# Autodesk Inventor assembly: Estructura_bk03
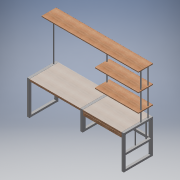
[picture p0: Inventor's stored thumbnail of the model, 180x180]
Saved by Autodesk Inventor 2016 (Build 200138000, 138)
## iProperties
Created: 2018-06-24
Part Number: Estructura_bk03
Document SubType Name: Weldment
Designer: damia
Weld Material: Iron, Cast
Mass: 65449.7 g
Surface Area: 113018 cm^2
Volume: 51991 cm^3
Density: 1.25887 g/cm^3
_SolveAssemblyDoc: Frame Generator Solve Assembly
_Version: 15.0.0
Author: damia
## Documents named in this file (12)
- C:\Users\damia\Documents\Inventor\escritorio_Damian\Estructura_bk03.iam
- C:\Users\damia\Documents\Inventor\Escritorio_Damian\Esqueleto.ipt
- C:\Users\damia\Documents\Inventor\Escritorio_Damian\Estructura\Frame\Frame0002.iam
- C:\Users\damia\Documents\Inventor\Escritorio_Damian\Part42.ipt
- C:\Users\damia\Documents\Inventor\Escritorio_Damian\VidrioChico.ipt
- C:\Users\damia\Documents\Inventor\Escritorio_Damian\tablero_chico.ipt
- C:\Users\damia\Documents\Inventor\Escritorio_Damian\tablero_granded.ipt
- C:\Users\damia\Documents\Inventor\Escritorio_Damian\Esqueleto_Estantes.ipt
- C:\Users\damia\Documents\Inventor\Escritorio_Damian\Estante01.ipt
- C:\Users\damia\Documents\Inventor\Escritorio_Damian\estante02.ipt
- C:\Users\damia\Documents\Inventor\Escritorio_Damian\FrenteChico.ipt
- C:\Users\damia\Documents\Inventor\Escritorio_Damian\FrenteGrande.ipt
## Components (13 placed, 11 different names)
1. Esqueleto:1 — Mate:1, Mate:2
2. Frame0002:1 [sub-assembly] — Flush:7, Flush:8, Flush:9, Mate:7, Flush:12, Mate:9
3. tablero_granded:1
4. tablero_chico:1
5. VidrioGrande:1
6. VidrioChico:1
7. Esqueleto_Estantes:1 — Flush:7, Flush:8
8. Estante01:1 — Flush:9, Flush:10, Flush:11
9. Estante01:2 — Flush:10, Flush:11, Mate:7
10. estante02:1 — Flush:12
11. FrenteChico:1 — Mate:10
12. FrenteGrande:1 — Flush:13, Mate:8, Mate:9, Mate:10
13. FrenteGrande:2 — Flush:13, Mate:8
## Relationships (23: Flush 13, Mate 10)
- Mate:1: Esqueleto:1
- Mate:2: Esqueleto:1
- [Flush]: tablero_granded:1 ↔ VidrioGrande:1
- [Flush]: tablero_granded:1 ↔ VidrioGrande:1
- [Flush]: tablero_chico:1 ↔ VidrioChico:1
- [Flush]: tablero_chico:1 ↔ VidrioChico:1
- [Flush]: Frame0002:1 ↔ tablero_chico:1
- [Mate]: Frame0002:1 ↔ tablero_chico:1
- [Mate]: Frame0002:1 ↔ tablero_chico:1
- [Mate]: Frame0002:1 ↔ tablero_granded:1
- [Flush]: Frame0002:1 ↔ tablero_granded:1
- [Mate]: Frame0002:1 ↔ tablero_granded:1
- Flush:7: Frame0002:1 ↔ Esqueleto_Estantes:1
- Flush:8: Frame0002:1 ↔ Esqueleto_Estantes:1
- Flush:9: Frame0002:1 ↔ Estante01:1
- Flush:10: Estante01:1 ↔ Estante01:2
- Flush:11: Estante01:1 ↔ Estante01:2
- Mate:7: Frame0002:1 ↔ Estante01:2
- Flush:12: Frame0002:1 ↔ estante02:1
- Flush:13: FrenteGrande:1 ↔ FrenteGrande:2
- Mate:8 (5 mm): FrenteGrande:1 ↔ FrenteGrande:2
- Mate:9 (5 mm): Frame0002:1 ↔ FrenteGrande:1
- Mate:10 (5 mm): FrenteChico:1 ↔ FrenteGrande:1
## Named parameters: d14_d8 = 0 mm, d16_d6 = 0 mm, d17_d7 = 0 mm, Altura = 700 mm, Profundidad = 600 mm, TablaAltura = 40 mm, CajonAltura = 370 mm, Largo = 2000 mm, d5_1 = 600 mm, CajonAncho = 900 mm, Cajon02Altura = 150 mm, Cajon01Altura = 55 mm, d11_1 = 900 mm
